# Autodesk Inventor assembly: joint2_inertia
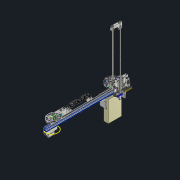
[picture p0: Inventor's stored thumbnail of the model, 180x180]
Saved by Autodesk Inventor 2022 (Build 260153000, 153)
## iProperties
Created: 2021-10-09
Part Number: joint2_inertia
Document SubType Name: Assembly
Designer: Yuta Kage
Mass: 13697.5 g
Surface Area: 28580.4 cm^2
Volume: 4985.75 cm^3
Density: 2.74732 g/cm^3
Author: Yuta Kage
## Documents named in this file (6)
- C:\Users\yuta0\Documents\GitHub\catchrobo_hardware\assy-scara\joint2_inertia.iam
- C:\Users\yuta0\Documents\GitHub\catchrobo_hardware\assy-scara\s-assy-linear_joint.iam
- C:\Users\yuta0\Documents\GitHub\catchrobo_hardware\assy-scara\s-assy-scara_link2.iam
- C:\Users\yuta0\Documents\GitHub\catchrobo_hardware\assy-scara\s-assy-scara-link4.iam
- C:\Users\yuta0\Documents\GitHub\catchrobo_hardware\assy-scara\s-assy-gripper.iam
- C:\Users\yuta0\Documents\GitHub\catchrobo_hardware\assy-scara\bisco.ipt
## Components (6 placed, 5 different names)
1. s-assy-scara_link2:1 [sub-assembly] — 角度:3, メイト:40, メイト:41, メイト:43
2. s-assy-linear_joint:1 [sub-assembly] — 角度:3, メイト:33, メイト:34, フラッシュ:1, メイト:40, メイト:41
3. s-assy-scara-link4:1 [sub-assembly] — メイト:33, メイト:34, フラッシュ:1, メイト:35, メイト:36, メイト:37
4. s-assy-gripper:1 [sub-assembly] — メイト:35, メイト:36, メイト:37, メイト:42, フラッシュ:2, フラッシュ:3
5. bisco:1 — メイト:42, フラッシュ:2, フラッシュ:3
6. bisco:2
## Component patterns: (2 elements, first: bisco:1)
## Relationships (13: Mate 9, Flush 3, Angle 1)
- 角度:3 [Angle] (180 deg): s-assy-scara_link2:1 ↔ s-assy-linear_joint:1
- フラッシュ:1 [Flush]: s-assy-linear_joint:1 ↔ s-assy-scara-link4:1
- メイト:33 [Mate]: s-assy-linear_joint:1 ↔ s-assy-scara-link4:1
- メイト:34 [Mate]: s-assy-linear_joint:1 ↔ s-assy-scara-link4:1
- メイト:35 [Mate]: s-assy-scara-link4:1 ↔ s-assy-gripper:1
- メイト:36 [Mate]: s-assy-scara-link4:1 ↔ s-assy-gripper:1
- メイト:37 [Mate]: s-assy-scara-link4:1 ↔ s-assy-gripper:1
- メイト:40 [Mate]: s-assy-scara_link2:1 ↔ s-assy-linear_joint:1
- メイト:41 [Mate]: s-assy-scara_link2:1 ↔ s-assy-linear_joint:1
- メイト:42 [Mate]: s-assy-gripper:1 ↔ bisco:1
- フラッシュ:2 [Flush] (5.5 mm): s-assy-gripper:1 ↔ bisco:1
- フラッシュ:3 [Flush]: s-assy-gripper:1 ↔ bisco:1
- メイト:43 [Mate]: s-assy-scara_link2:1
